# Autodesk Inventor assembly: AssembledFeederStation
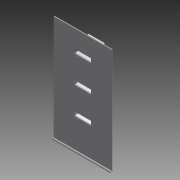
[picture p0: Inventor's stored thumbnail of the model, 180x180]
Saved by Autodesk Inventor 2011 SP1 (Build 150282100, 282)
## iProperties
Created: 2013-01-18
Part Number: AssembledFeederStation
Document SubType Name: Assembly
Designer: wes
Author: wes
## Documents named in this file (4)
- F:\ALL FILES\My Documents\GitHub\2013CAD\2013 robot\CurvedShooter\feederStation\AssembledFeederStation.iam
- F:\ALL FILES\My Documents\GitHub\2013CAD\2013 robot\CurvedShooter\feederStation\feederStationSlots.ipt
- F:\ALL FILES\My Documents\GitHub\2013CAD\2013 robot\CurvedShooter\feederStation\slideFeeder.ipt
- F:\ALL FILES\My Documents\GitHub\2013CAD\2013 robot\CurvedShooter\feederStation\1in bolt.ipt
## Components (10 placed, 3 different names)
1. feederStationSlots:1 — Insert:1, Insert:2, Insert:3, Insert:4, Insert:5, Insert:6, Insert:7, Insert:8, Insert:9, Insert:10, Insert:11, Insert:12
2. slideFeeder:1 — Insert:3, Insert:4
3. slideFeeder:2 — Insert:9, Insert:10
4. slideFeeder:3 — Insert:11, Insert:12
5. 1in bolt:1 — Insert:1
6. 1in bolt:2 — Insert:2
7. 1in bolt:3 — Insert:6
8. 1in bolt:4 — Insert:5
9. 1in bolt:5 — Insert:7
10. 1in bolt:6 — Insert:8
## Relationships (12: Insert 12)
- Insert:1: feederStationSlots:1 ↔ 1in bolt:1
- Insert:2: feederStationSlots:1 ↔ 1in bolt:2
- Insert:3: feederStationSlots:1 ↔ slideFeeder:1
- Insert:4: feederStationSlots:1 ↔ slideFeeder:1
- Insert:5: feederStationSlots:1 ↔ 1in bolt:4
- Insert:6: feederStationSlots:1 ↔ 1in bolt:3
- Insert:7: feederStationSlots:1 ↔ 1in bolt:5
- Insert:8: feederStationSlots:1 ↔ 1in bolt:6
- Insert:9: feederStationSlots:1 ↔ slideFeeder:2
- Insert:10: feederStationSlots:1 ↔ slideFeeder:2
- Insert:11: feederStationSlots:1 ↔ slideFeeder:3
- Insert:12: feederStationSlots:1 ↔ slideFeeder:3
